# Autodesk Inventor assembly: Print
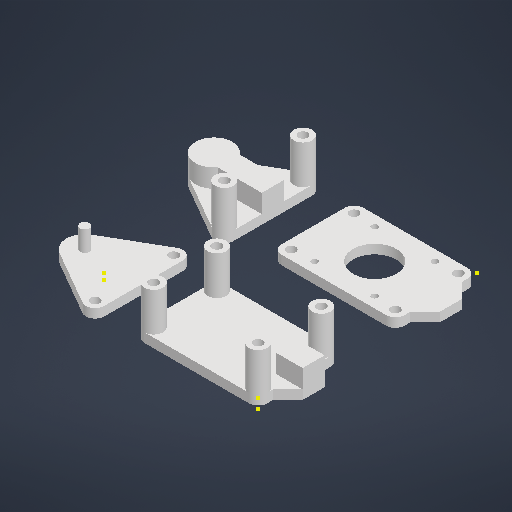
[picture p0: Inventor's stored thumbnail of the model, 512x512]
Saved by Autodesk Inventor 2026 (Build 300175000, 175)
## iProperties
Created: 2025-04-17
Part Number: Print
Document SubType Name: Assembly
Designer: sdcel
Author: sdcel
## Documents named in this file (5)
- C:\Users\sdcel\OneDrive\Documents\College_Work\3rd_Year\2025_Spring\CSCE_462_503\Automatic_Curtain\Models\Print.iam
- C:\Users\sdcel\OneDrive\Documents\College_Work\3rd_Year\2025_Spring\CSCE_462_503\Automatic_Curtain\Models\EndTop3.ipt
- C:\Users\sdcel\OneDrive\Documents\College_Work\3rd_Year\2025_Spring\CSCE_462_503\Automatic_Curtain\Models\MotorBot.ipt
- C:\Users\sdcel\OneDrive\Documents\College_Work\3rd_Year\2025_Spring\CSCE_462_503\Automatic_Curtain\Models\MotorTop.ipt
- C:\Users\sdcel\OneDrive\Documents\College_Work\3rd_Year\2025_Spring\CSCE_462_503\Automatic_Curtain\Models\End.ipt
## Components (4 placed, 4 different names)
1. EndTop3:1 — Mate:4
2. MotorBot:1 — Mate:2
3. MotorTop:1 — Mate:1
4. End:1 — Mate:3
## Relationships (4: Mate 4)
- Mate:1: MotorTop:1
- Mate:2: MotorBot:1
- Mate:3: End:1
- Mate:4: EndTop3:1
